# Autodesk Inventor assembly: Assembly_Cube_LED_Matrix_v2
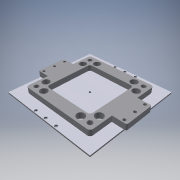
[picture p0: Inventor's stored thumbnail of the model, 180x180]
Saved by Autodesk Inventor 2019 (Build 230136000, 136)
## iProperties
Created: 2018-05-19
Part Number: Assembly_Cube_LED_Matrix_v2
Material: Generisch
Document SubType Name: Assembly
Designer: diederichbenedict
Mass: 63.6464 g
Surface Area: 536.97 cm^2
Volume: 62.4487 cm^3
Density: 1.01918 g/cm^3
Author: diederichbenedict
## Documents named in this file (3)
- C:\Users\marsikovabarbora\Dropbox\UC2\02_CAD\INVENTOR\uc2_v3\Assembly_Cube_LED_Matrix_8x8_v3.iam
- C:\Users\marsikovabarbora\Dropbox\UC2\02_CAD\INVENTOR\uc2_v3\30_IM_LED_holder_8x8_v3.ipt
- C:\Users\marsikovabarbora\Dropbox\UC2\02_CAD\INVENTOR\uc2_v3\00_LED-ARRAY.ipt
## Components (2 placed, 2 different names)
1. 30_IM_LED_holder_8x8_v3:1 — Passend:1, Passend:2, Passend:3, Mate:4, Mate:5
2. 00_LED-ARRAY:1 — Mate:4, Mate:5
## Relationships (5: Mate 5)
- Passend:1 [Mate]: 30_IM_LED_holder_8x8_v3:1
- Passend:2 [Mate]: 30_IM_LED_holder_8x8_v3:1
- Passend:3 [Mate]: 30_IM_LED_holder_8x8_v3:1
- Mate:4: 30_IM_LED_holder_8x8_v3:1 ↔ 00_LED-ARRAY:1
- Mate:5: 30_IM_LED_holder_8x8_v3:1 ↔ 00_LED-ARRAY:1
